# Autodesk Inventor assembly: リンク_6_1
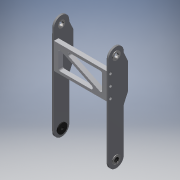
[picture p0: Inventor's stored thumbnail of the model, 180x180]
Saved by Autodesk Inventor 2018 (Build 220112000, 112)
## iProperties
Created: 2016-08-23
Part Number: リンク_6_1
Material: 一般
Document SubType Name: Assembly
Designer: hiro
Mass: 25.265 g
Surface Area: 146.992 cm^2
Volume: 11.3922 cm^3
Density: 2.21774 g/cm^3
Author: hiro
## Documents named in this file (5)
- C:\Users\taka\Documents\github\OpenPlatform\mechanism\OpenPlatform_ver3_0\下半身_160823\リンク\リンク_6_3.iam
- C:\Users\taka\Documents\github\OpenPlatform\mechanism\OpenPlatform_ver3_0\既製品\NSK_RB_MF85ZZ\MF85ZZ.iam
- C:\Users\taka\Documents\github\OpenPlatform\mechanism\OpenPlatform_ver3_0\下半身\リンク\ふくらはぎ\リンク_ふくらはぎ_サブフレーム_1_2(予備案).ipt
- C:\Users\taka\Documents\github\OpenPlatform\mechanism\OpenPlatform_ver3_0\下半身\リンク\スペーサ\足首_スペーサ_1_1.ipt
- C:\Users\taka\Documents\github\OpenPlatform\mechanism\OpenPlatform_ver3_0\下半身_160823\リンク\リンク_メインフレーム_6_3.ipt
## Components (9 placed, 4 different names)
1. MF85ZZ:1 [sub-assembly] — 挿入:9
2. MF85ZZ:2 [sub-assembly] — 挿入:10
3. MF85ZZ:3 [sub-assembly] — 挿入:8
4. MF85ZZ:4 [sub-assembly] — 挿入:7
5. リンク_ふくらはぎ_サブフレーム_1_2(予備案):1 — 挿入:1, 挿入:2, 挿入:3, 挿入:4
6. 足首_スペーサ_1_1:1 — 挿入:5
7. 足首_スペーサ_1_1:2 — 挿入:6
8. リンク_メインフレーム_6_3:1 — 挿入:1, 挿入:2, 挿入:6, 挿入:7, 挿入:10
9. リンク_メインフレーム_6_3:2 — 挿入:3, 挿入:4, 挿入:5, 挿入:8, 挿入:9
## Relationships (10: Insert 10)
- 挿入:1 [Insert]: リンク_ふくらはぎ_サブフレーム_1_2(予備案):1 ↔ リンク_メインフレーム_6_3:1
- 挿入:2 [Insert]: リンク_ふくらはぎ_サブフレーム_1_2(予備案):1 ↔ リンク_メインフレーム_6_3:1
- 挿入:3 [Insert]: リンク_ふくらはぎ_サブフレーム_1_2(予備案):1 ↔ リンク_メインフレーム_6_3:2
- 挿入:4 [Insert]: リンク_ふくらはぎ_サブフレーム_1_2(予備案):1 ↔ リンク_メインフレーム_6_3:2
- 挿入:5 [Insert]: 足首_スペーサ_1_1:1 ↔ リンク_メインフレーム_6_3:2
- 挿入:6 [Insert]: 足首_スペーサ_1_1:2 ↔ リンク_メインフレーム_6_3:1
- 挿入:7 [Insert]: MF85ZZ:4 ↔ リンク_メインフレーム_6_3:1
- 挿入:8 [Insert]: MF85ZZ:3 ↔ リンク_メインフレーム_6_3:2
- 挿入:9 [Insert]: MF85ZZ:1 ↔ リンク_メインフレーム_6_3:2
- 挿入:10 [Insert]: MF85ZZ:2 ↔ リンク_メインフレーム_6_3:1
